# Autodesk Inventor assembly: EstructuraRPegante
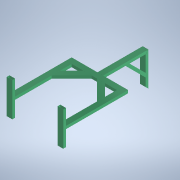
[picture p0: Inventor's stored thumbnail of the model, 180x180]
Saved by Autodesk Inventor 2021 (Build 250183000, 183)
## iProperties
Created: 2021-06-11
Part Number: EstructuraRPegante
Document SubType Name: Assembly
Designer: lcper
Author: lcper
## Documents named in this file (8)
- C:\UNal\S10\Robotica\Proyecto\EstructuraRPegante.iam
- C:\UNal\S10\Robotica\Proyecto\PerfilH1.ipt
- C:\UNal\S10\Robotica\Proyecto\PerfilV1.ipt
- C:\UNal\S10\Robotica\Proyecto\PerfilV2.ipt
- C:\UNal\S10\Robotica\Proyecto\PerfilH2.ipt
- C:\UNal\S10\Robotica\Proyecto\PerfilH34.ipt
- C:\UNal\S10\Robotica\Proyecto\PerfilD1.ipt
- C:\UNal\S10\Robotica\Proyecto\PerfilD2.ipt
## Components (10 placed, 7 different names)
1. PerfilH1:1 — Mate:1, Mate:2, Mate:3, Mate:4, Mate:5, Mate:6, Mate:7, Mate:8, Mate:17, Mate:19, Mate:21, Mate:22
2. PerfilV1:1 — Mate:6, Mate:7, Mate:8, Mate:9, Mate:10, Mate:24
3. PerfilV2:1 — Mate:1, Mate:2, Mate:3, Mate:12, Mate:15, Mate:16, Mate:18
4. PerfilV2:2 — Mate:4, Mate:5, Mate:11, Mate:13, Mate:14, Mate:20
5. PerfilH2:1 — Mate:9, Mate:10, Mate:23, Mate:25
6. PerfilH34:1 — Mate:11, Mate:13, Mate:14
7. PerfilH34:2 — Mate:12, Mate:15, Mate:16
8. PerfilD1:1 — Mate:17, Mate:18, Mate:19
9. PerfilD1:2 — Mate:20, Mate:21, Mate:22
10. PerfilD2:1 — Mate:23, Mate:24, Mate:25
## Relationships (25: Mate 25)
- Mate:1: PerfilH1:1 ↔ PerfilV2:1
- Mate:2: PerfilH1:1 ↔ PerfilV2:1
- Mate:3: PerfilH1:1 ↔ PerfilV2:1
- Mate:4: PerfilH1:1 ↔ PerfilV2:2
- Mate:5: PerfilH1:1 ↔ PerfilV2:2
- Mate:6: PerfilH1:1 ↔ PerfilV1:1
- Mate:7: PerfilH1:1 ↔ PerfilV1:1
- Mate:8: PerfilH1:1 ↔ PerfilV1:1
- Mate:9: PerfilV1:1 ↔ PerfilH2:1
- Mate:10: PerfilV1:1 ↔ PerfilH2:1
- Mate:11: PerfilV2:2 ↔ PerfilH34:1
- Mate:12: PerfilV2:1 ↔ PerfilH34:2
- Mate:13: PerfilV2:2 ↔ PerfilH34:1
- Mate:14: PerfilV2:2 ↔ PerfilH34:1
- Mate:15: PerfilV2:1 ↔ PerfilH34:2
- Mate:16: PerfilV2:1 ↔ PerfilH34:2
- Mate:17: PerfilH1:1 ↔ PerfilD1:1
- Mate:18: PerfilV2:1 ↔ PerfilD1:1
- Mate:19: PerfilH1:1 ↔ PerfilD1:1
- Mate:20: PerfilV2:2 ↔ PerfilD1:2
- Mate:21: PerfilH1:1 ↔ PerfilD1:2
- Mate:22: PerfilH1:1 ↔ PerfilD1:2
- Mate:23: PerfilH2:1 ↔ PerfilD2:1
- Mate:24: PerfilV1:1 ↔ PerfilD2:1
- Mate:25: PerfilH2:1 ↔ PerfilD2:1
